# Autodesk Inventor assembly: T04
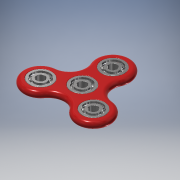
[picture p0: Inventor's stored thumbnail of the model, 180x180]
Saved by Autodesk Inventor 2018 (Build 220112000, 112)
## iProperties
Created: 2020-06-25
Part Number: T04
Document SubType Name: Assembly
Designer: Diego
Author: Diego
## Documents named in this file (4)
- D:\DocumentsWin\Inventor\ProjectName\T04.iam
- D:\DocumentsWin\Inventor\ProjectName\T04.ipt
- D:\DocumentsWin\Inventor\ProjectName\Assembly1\Design Accelerator\Bearing1.iam
- D:\DocumentsWin\Inventor\ProjectName\Assembly1\Design Accelerator\Bearing2.iam
## Components (5 placed, 2 different names)
1. T04:1 — Mate:1, Mate:2, Mate:3, Mate:4, Angle:1
2. Bearing:1 [sub-assembly] — Mate:1, Mate:2, Mate:5, Mate:7
3. Bearing:2 [sub-assembly] — Mate:3, Mate:4
4. Bearing:3 [sub-assembly]
5. Bearing:4 [sub-assembly]
## Component patterns: (3 elements, first: Bearing:2)
## Relationships (8: Mate 7, Angle 1)
- Mate:1: T04:1 ↔ Bearing:1
- Mate:2: T04:1 ↔ Bearing:1
- Mate:3: T04:1 ↔ Bearing:2
- Mate:4: T04:1 ↔ Bearing:2
- Mate:5: Bearing:1
- Mate:6
- Mate:7: Bearing:1
- Angle:1 (0 deg): T04:1
